# Autodesk Inventor assembly: Cycloidal Drive
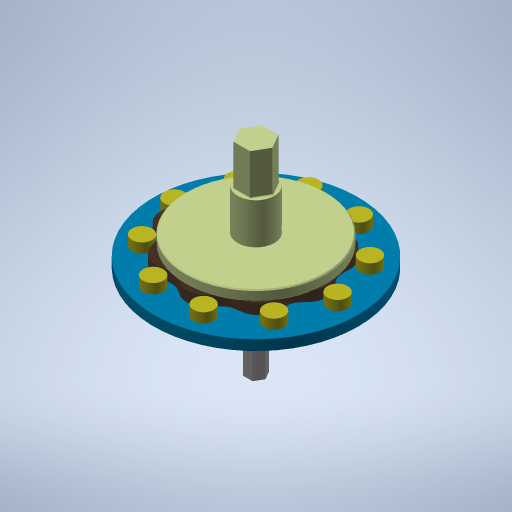
[picture p0: Inventor's stored thumbnail of the model, 512x512]
Saved by Autodesk Inventor 2023 (Build 270158000, 158)
## iProperties
Created: 2023-06-26
Part Number: Cycloidal Drive
Document SubType Name: Assembly
Designer: Normal
Mass: 727.575 g
Surface Area: 407.382 cm^2
Volume: 91.3804 cm^3
Density: 7.96204 g/cm^3
Author: rh4720
## Documents named in this file (6)
- C:\Users\Ranjini\OneDrive\Desktop\New folder\Assembly.iam
- cycloidaldrive.iam
- C:\Users\Ranjini\OneDrive\Desktop\New folder\Base.ipt
- C:\Users\Ranjini\OneDrive\Desktop\New folder\Input Shaft.ipt
- C:\Users\Ranjini\OneDrive\Desktop\New folder\Disk.ipt
- C:\Users\Ranjini\OneDrive\Desktop\New folder\Output Shaft.ipt
## Components (4 placed, 4 different names)
1. Base:1 — Einfügen:1, Einfügen:3, DRIVE_ME
2. Input Shaft:1 — Einfügen:1, Einfügen:2, DRIVE_ME
3. Disk:1 — Einfügen:2
4. Output Shaft:1 — Einfügen:3
## Relationships (4: Insert 3, Angle 1)
- Einfügen:1 [Insert]: Base:1 ↔ Input Shaft:1
- Einfügen:2 [Insert]: Input Shaft:1 ↔ Disk:1
- Einfügen:3 [Insert] (5 mm): Base:1 ↔ Output Shaft:1
- DRIVE_ME [Angle] (0 deg): Base:1 ↔ Input Shaft:1
